# Autodesk Inventor assembly: new_assembly_auger
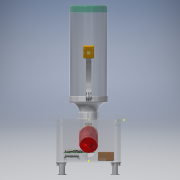
[picture p0: Inventor's stored thumbnail of the model, 180x180]
Saved by Autodesk Inventor 2019 (Build 230136000, 136)
## iProperties
Created: 2019-01-23
Part Number: new_assembly_auger
Document SubType Name: Assembly
Designer: jmc
Author: jmc
## Documents named in this file (10)
- C:\Users\l0086\Desktop\Models\CatFeeder\version4 (auger)\new_assembly_auger.iam
- C:\Users\l0086\Desktop\Models\CatFeeder\Case\version3\case_top.ipt
- C:\Users\l0086\Desktop\Models\CatFeeder\Case\version3\case_bottom.ipt
- C:\Users\l0086\Desktop\Models\CatFeeder\version4 (auger)\subassembly_auger_case.iam
- C:\Users\l0086\Desktop\Models\3party\Boards\ArduinoNano\arduino nano.iam
- C:\Users\l0086\Desktop\Models\3party\Boards\Raspberry Pi 3\Raspberry Pi 3.ipt
- C:\Users\l0086\Desktop\Models\3party\Trasformer\Transformer.ipt
- C:\Users\l0086\Desktop\Models\CatFeeder\Case\version3\pata_mod.ipt
- C:\Users\l0086\Desktop\Models\CatFeeder\Case\version2\pata_macho.ipt
- C:\Users\l0086\Desktop\Models\CatFeeder\version4 (auger)\subassembly_jar_jarcone_gopro.iam
## Components (15 placed, 9 different names)
1. subassembly_jar_jarcone_gopro:1 [sub-assembly] — Rotational:9
2. case_top:1 — Rigid:1, Rigid:3, Rotational:9
3. case_bottom:1 — Rigid:1, Mate:1, Mate:2, Mate:5, Mate:6, Mate:7, Mate:8, Mate:9
4. subassembly_auger_case:1 [sub-assembly] — Rigid:3
5. arduino nano:1 [sub-assembly] — Mate:5
6. Transformer:1 — Mate:1, Mate:2, Mate:4
7. Raspberry Pi 3:1 — Mate:4
8. pata_mod:1 — Mate:7, Rigid:4
9. pata_mod:2 — Mate:8, Rigid:7
10. pata_mod:3 — Mate:9, Rigid:6
11. pata_mod:4 — Mate:6, Rigid:5
12. pata_macho:1 — Rigid:4
13. pata_macho:2 — Rigid:5
14. pata_macho:3 — Rigid:7
15. pata_macho:4 — Rigid:6
## Relationships (15: Mate 8, WeldJoint 6, RevoluteJoint 1)
- Rigid:1 [WeldJoint]: case_top:1 ↔ case_bottom:1
- Rigid:3 [WeldJoint]: case_top:1 ↔ subassembly_auger_case:1
- Mate:1 (1 mm): case_bottom:1 ↔ Transformer:1
- Mate:2: case_bottom:1 ↔ Transformer:1
- Mate:4 (-2 mm): Transformer:1 ↔ Raspberry Pi 3:1
- Mate:5 (10 mm): case_bottom:1 ↔ arduino nano:1
- Mate:6: case_bottom:1 ↔ pata_mod:4
- Mate:7: case_bottom:1 ↔ pata_mod:1
- Mate:8: case_bottom:1 ↔ pata_mod:2
- Mate:9: case_bottom:1 ↔ pata_mod:3
- Rigid:4 [WeldJoint]: pata_mod:1 ↔ pata_macho:1
- Rigid:5 [WeldJoint]: pata_mod:4 ↔ pata_macho:2
- Rigid:6 [WeldJoint]: pata_mod:3 ↔ pata_macho:4
- Rigid:7 [WeldJoint]: pata_mod:2 ↔ pata_macho:3
- Rotational:9 [RevoluteJoint]: subassembly_jar_jarcone_gopro:1 ↔ case_top:1
